# Autodesk Inventor assembly: block
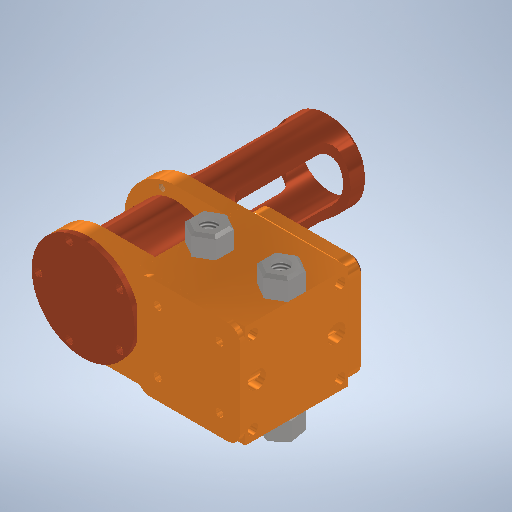
[picture p0: Inventor's stored thumbnail of the model, 512x512]
Saved by Autodesk Inventor 2025.1 (Build 291241000, 241)
## iProperties
Created: 2024-09-18
Part Number: block
Document SubType Name: Assembly
Designer: ffogue
Author: ffogue
## Documents named in this file (15)
- C:\Users\ffogue\Documents\Inventor\Cylinder Radial Steam Engine\block.iam
- C:\Users\ffogue\Documents\Inventor\Cylinder Radial Steam Engine\23.ipt
- C:\Users\ffogue\Documents\Inventor\Cylinder Radial Steam Engine\26.ipt
- C:\Users\ffogue\Documents\Inventor\Cylinder Radial Steam Engine\27.ipt
- C:\Users\ffogue\Documents\Inventor\Cylinder Radial Steam Engine\26A.ipt
- C:\Users\ffogue\Documents\Inventor\Cylinder Radial Steam Engine\34.ipt
- C:\Users\ffogue\Documents\Inventor\Cylinder Radial Steam Engine\35.ipt
- C:\Users\ffogue\Documents\Inventor\Cylinder Radial Steam Engine\32.ipt
- C:\Users\ffogue\Documents\Inventor\Cylinder Radial Steam Engine\49.ipt
- C:\Users\ffogue\Documents\Inventor\Cylinder Radial Steam Engine\50.ipt
- C:\Users\ffogue\Documents\Inventor\Cylinder Radial Steam Engine\36.ipt
- C:\Users\ffogue\Documents\Inventor\Cylinder Radial Steam Engine\38.ipt
- C:\Users\ffogue\Documents\Inventor\Cylinder Radial Steam Engine\39.ipt
- C:\Users\ffogue\Documents\Inventor\Cylinder Radial Steam Engine\29.ipt
- C:\Users\ffogue\Documents\Inventor\Cylinder Radial Steam Engine\28.ipt
## Components (21 placed, 14 different names)
1. 23:1 — Mate:1, Mate:2, Mate:3, Mate:4, Insert:3, Mate:5, Mate:6, Mate:10, Mate:11, Mate:12, Mate:13, Insert:7, Insert:8, Mate:14, Insert:13, Insert:14, Insert:15, Insert:16
2. 26:1 — Mate:3, Insert:7
3. 27:1 — Mate:1, Mate:2, Insert:8, Insert:18
4. 26A:1 — Mate:4, Insert:3, Insert:4, Insert:5
5. 34:1 — Mate:5, Insert:5, Mate:9
6. 34:2 — Mate:6, Insert:4, Mate:7, Mate:8, Insert:6, Mate:20
7. 35:1 — Mate:7, Mate:8, Insert:6, Cylindrical:1
8. 32:1 — Mate:9, Cylindrical:1, Mate:15, Mate:16, Mate:17, Mate:20
9. 49:1 — Mate:13, Insert:9, Insert:15
10. 49:2 — Mate:10, Insert:10, Insert:16
11. 49:3 — Mate:12, Insert:11, Insert:14
12. 49:4 — Mate:11, Insert:12, Insert:13
13. 50:1 — Insert:11
14. 50:2 — Insert:12, Mate:14
15. 50:3 — Insert:9
16. 50:4 — Insert:10
17. 36:1 — Mate:15, Mate:16, Flush:1
18. 38:1 — Mate:17, Mate:19, Insert:17
19. 39:1 — Mate:19, Insert:17, Flush:1
20. 29:1 — Insert:18, Mate:21, Insert:19
21. 28:1 — Mate:21, Insert:19
## Relationships (39: Mate 20, Insert 17, CylindricalJoint 1, Flush 1)
- Mate:1: 23:1 ↔ 27:1
- Mate:2: 23:1 ↔ 27:1
- Mate:3: 23:1 ↔ 26:1
- Mate:4: 23:1 ↔ 26A:1
- Insert:3: 23:1 ↔ 26A:1
- Mate:5: 23:1 ↔ 34:1
- Mate:6: 23:1 ↔ 34:2
- Insert:4: 26A:1 ↔ 34:2
- Insert:5: 26A:1 ↔ 34:1
- Mate:7: 34:2 ↔ 35:1
- Mate:8: 34:2 ↔ 35:1
- Insert:6: 34:2 ↔ 35:1
- Mate:9: 34:1 ↔ 32:1
- Cylindrical:1: 35:1 ↔ 32:1
- Mate:10: 23:1 ↔ 49:2
- Mate:11: 23:1 ↔ 49:4
- Mate:12: 23:1 ↔ 49:3
- Mate:13: 23:1 ↔ 49:1
- Insert:7: 23:1 ↔ 26:1
- Insert:8: 23:1 ↔ 27:1
- Insert:9: 49:1 ↔ 50:3
- Insert:10: 49:2 ↔ 50:4
- Insert:11: 49:3 ↔ 50:1
- Insert:12: 49:4 ↔ 50:2
- Mate:14: 23:1 ↔ 50:2
- Insert:13 (-15.8 mm): 23:1 ↔ 49:4
- Insert:14 (-15.8 mm): 23:1 ↔ 49:3
- Insert:15 (-15.8 mm): 23:1 ↔ 49:1
- Insert:16 (-15.8 mm): 23:1 ↔ 49:2
- Mate:15: 32:1 ↔ 36:1
- Mate:16: 32:1 ↔ 36:1
- Mate:17: 32:1 ↔ 38:1
- Mate:19: 38:1 ↔ 39:1
- Insert:17: 38:1 ↔ 39:1
- Mate:20: 34:2 ↔ 32:1
- Flush:1: 36:1 ↔ 39:1
- Insert:18: 27:1 ↔ 29:1
- Mate:21: 29:1 ↔ 28:1
- Insert:19 (-6 mm): 29:1 ↔ 28:1
